# Autodesk Inventor assembly: s-assy-shooter_unit
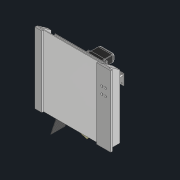
[picture p0: Inventor's stored thumbnail of the model, 180x180]
Saved by Autodesk Inventor 2021 (Build 250183000, 183)
## iProperties
Created: 2021-08-20
Part Number: s-assy-shooter_unit
Document SubType Name: Assembly
Designer: yuta0
Author: yuta0
## Documents named in this file (13)
- C:\Users\yuta0\Documents\GitHub\catchrobo_hardware\assy-shooter\s-assy-shooter_unit.iam
- C:\Users\yuta0\Documents\GitHub\catchrobo_hardware\assy-shooter\s_carbon_plate1.ipt
- C:\Users\yuta0\Documents\GitHub\catchrobo_hardware\assy-robot\MG_996R.iam
- C:\Users\yuta0\Documents\GitHub\catchrobo_hardware\assy-shooter\s_base3.ipt
- C:\Users\yuta0\Documents\GitHub\catchrobo_hardware\assy-shooter\CB3-25.ipt
- C:\Users\yuta0\Documents\GitHub\catchrobo_hardware\assy-shooter\s_carbon_plate2.ipt
- C:\Users\yuta0\Documents\GitHub\catchrobo_hardware\assy-shooter\s_base2.ipt
- C:\Users\yuta0\Documents\GitHub\catchrobo_hardware\assy-shooter\s_carbon_plate3.ipt
- C:\Users\yuta0\Documents\GitHub\catchrobo_hardware\assy-shooter\s_base4.ipt
- C:\Users\yuta0\Downloads\新しいフォルダー\bisco.ipt
- C:\Users\yuta0\Documents\GitHub\catchrobo_hardware\assy-robot\CBSTNR3-12.ipt
- C:\Users\yuta0\Documents\GitHub\catchrobo_hardware\assy-robot\ARF-410E.ipt
- C:\Users\yuta0\Documents\GitHub\catchrobo_hardware\assy-robot\ARF-420E.ipt
## Components (15 placed, 12 different names)
1. s_carbon_plate1:1 — メイト:13, メイト:14, メイト:20, メイト:21, メイト:23, フラッシュ:5, フラッシュ:6
2. s_base3:1 — メイト:11, 角度:1, メイト:22, メイト:24, メイト:25, メイト:26, メイト:27, メイト:28, メイト:29, メイト:30
3. CB3-25:1 — メイト:26, メイト:27
4. s_carbon_plate2:1 — メイト:11, 角度:1, メイト:24, メイト:25, メイト:34
5. s_base2:1 — メイト:13, メイト:14, フラッシュ:5, メイト:35, メイト:36, メイト:37, メイト:38
6. s_carbon_plate3:1 — メイト:15, メイト:16, メイト:17, フラッシュ:4, メイト:31, メイト:35, メイト:36, メイト:39
7. MG_996R:2 [sub-assembly] — メイト:15, メイト:16, メイト:17, メイト:22, メイト:28, メイト:32
8. s_base4:1 — メイト:20, メイト:21, フラッシュ:4, フラッシュ:6
9. bisco:1 — メイト:23, メイト:34
10. ARF-410E:1 — メイト:31, メイト:32
11. ARF-420E:1 — メイト:37, メイト:38, メイト:39
12. CBSTNR3-12:1 — メイト:29, メイト:30
13. CBSTNR3-12:2
14. CBSTNR3-12:3
15. CBSTNR3-12:4
## Component patterns: (4 elements, first: CBSTNR3-12:1)
## Relationships (29: Mate 25, Flush 3, Angle 1)
- メイト:11 [Mate]: s_base3:1 ↔ s_carbon_plate2:1
- 角度:1 [Angle] (180 deg): s_base3:1 ↔ s_carbon_plate2:1
- メイト:13 [Mate]: s_carbon_plate1:1 ↔ s_base2:1
- メイト:14 [Mate]: s_carbon_plate1:1 ↔ s_base2:1
- メイト:15 [Mate]: s_carbon_plate3:1 ↔ MG_996R:2
- メイト:16 [Mate]: s_carbon_plate3:1 ↔ MG_996R:2
- メイト:17 [Mate] (10 mm): s_carbon_plate3:1 ↔ MG_996R:2
- メイト:20 [Mate]: s_carbon_plate1:1 ↔ s_base4:1
- メイト:21 [Mate]: s_carbon_plate1:1 ↔ s_base4:1
- フラッシュ:4 [Flush]: s_carbon_plate3:1 ↔ s_base4:1
- メイト:22 [Mate]: s_base3:1 ↔ MG_996R:2
- メイト:23 [Mate]: s_carbon_plate1:1 ↔ bisco:1
- メイト:24 [Mate]: s_base3:1 ↔ s_carbon_plate2:1
- メイト:25 [Mate]: s_base3:1 ↔ s_carbon_plate2:1
- メイト:26 [Mate]: s_base3:1 ↔ CB3-25:1
- メイト:27 [Mate]: s_base3:1 ↔ CB3-25:1
- メイト:28 [Mate]: s_base3:1 ↔ MG_996R:2
- メイト:29 [Mate]: s_base3:1 ↔ CBSTNR3-12:1
- メイト:30 [Mate]: s_base3:1 ↔ CBSTNR3-12:1
- メイト:31 [Mate]: s_carbon_plate3:1 ↔ ARF-410E:1
- メイト:32 [Mate]: MG_996R:2 ↔ ARF-410E:1
- メイト:34 [Mate]: s_carbon_plate2:1 ↔ bisco:1
- フラッシュ:5 [Flush]: s_carbon_plate1:1 ↔ s_base2:1
- フラッシュ:6 [Flush]: s_carbon_plate1:1 ↔ s_base4:1
- メイト:35 [Mate]: s_base2:1 ↔ s_carbon_plate3:1
- メイト:36 [Mate]: s_base2:1 ↔ s_carbon_plate3:1
- メイト:37 [Mate]: s_base2:1 ↔ ARF-420E:1
- メイト:38 [Mate]: s_base2:1 ↔ ARF-420E:1
- メイト:39 [Mate]: s_carbon_plate3:1 ↔ ARF-420E:1
